# Autodesk Inventor assembly: Motorhalterung_Foerderband.ipt
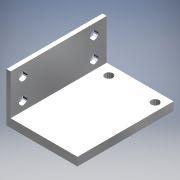
[picture p0: Inventor's stored thumbnail of the model, 180x180]
Saved by Autodesk Inventor 2018 (Build 220112000, 112)
## iProperties
Created: 2018-03-26
Part Number: Motorhalterung_Foerderband.ipt
Material: Generisch
Document SubType Name: Assembly
Designer: Julian
Author: Julian
## Documents named in this file (3)
- C:\Users\Julian\Desktop\Schule\5AHME\Diplomarbeit\Git\fuettr_prototype\Mechanical\Inventorskizzen\Motorhalterung_Foerderband.ipt.iam
- C:\Users\Julian\Desktop\Schule\5AHME\Diplomarbeit\Git\fuettr_prototype\Mechanical\Inventorskizzen\Motorhalterung_Grundplatte.ipt
- C:\Users\Julian\Desktop\Schule\5AHME\Diplomarbeit\Git\fuettr_prototype\Mechanical\Inventorskizzen\Motorhalterung_Stützleiste.ipt
## Components (2 placed, 2 different names)
1. Motorhalterung_Grundplatte:1 — Starr:2
2. Motorhalterung_Stützleiste:1 — Starr:2
## Relationships (1: WeldJoint 1)
- Starr:2 [WeldJoint]: Motorhalterung_Grundplatte:1 ↔ Motorhalterung_Stützleiste:1
